# Autodesk Inventor assembly: Assembly1
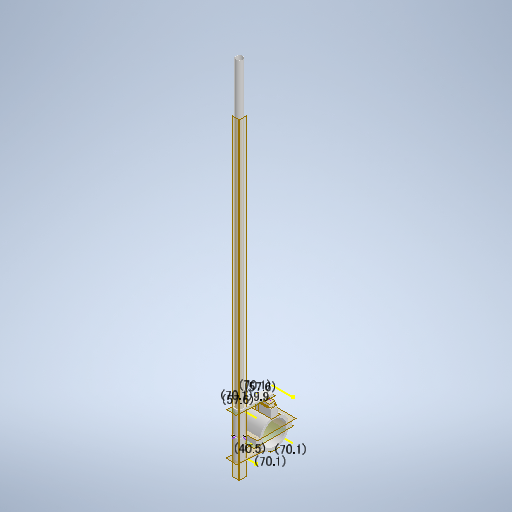
[picture p0: Inventor's stored thumbnail of the model, 512x512]
Saved by Autodesk Inventor 2025.2 (Build 292293000, 293)
## iProperties
Created: 2024-12-15
Part Number: Assembly1
Document SubType Name: Assembly
Designer: mahhy
Mass: 1247.47 g
Surface Area: 2591.78 cm^2
Volume: 1247.47 cm^3
Density: 1 g/cm^3
Author: mahhy
## Documents named in this file (15)
- D:\兵庫県立大\鳥人間部\尾翼データ\Assembly1.iam
- D:\兵庫県立大\鳥人間部\尾翼データ\motor_mount1.ipt
- D:\兵庫県立大\鳥人間部\尾翼データ\motor_mount2.ipt
- D:\兵庫県立大\鳥人間部\尾翼データ\wing1.ipt
- D:\兵庫県立大\鳥人間部\尾翼データ\bearing.ipt
- D:\兵庫県立大\鳥人間部\尾翼データ\arm1.ipt
- D:\兵庫県立大\鳥人間部\尾翼データ\arm2.ipt
- D:\兵庫県立大\鳥人間部\尾翼データ\servo_motor.ipt
- D:\兵庫県立大\鳥人間部\尾翼データ\pole.ipt
- D:\兵庫県立大\鳥人間部\尾翼データ\Assembly1\AIP\FEA\ewx9ztyo0.fins
- D:\兵庫県立大\鳥人間部\尾翼データ\Assembly1\AIP\FEA\ewx9ztyo0.fsat
- D:\兵庫県立大\鳥人間部\尾翼データ\Assembly1\AIP\FEA\ewx9ztyo0.ftes
- D:\兵庫県立大\鳥人間部\尾翼データ\Assembly1\AIP\FEA\ewx9ztyo0.fwiz
- D:\兵庫県立大\鳥人間部\尾翼データ\Assembly1\AIP\FEA\ewx9ztyrk.fmsh
- D:\兵庫県立大\鳥人間部\尾翼データ\Assembly1\AIP\FEA\ewx9ztyrl.fres
## Components (8 placed, 8 different names)
1. motor_mount1:1 — リジッド:1, リジッド:2
2. motor_mount2:1 — リジッド:1, 挿入:4
3. wing1:1 — 挿入:3, 挿入:5
4. bearing:1 — 挿入:1, 挿入:4
5. arm1:2 — 挿入:3, メイト:1
6. arm2:2 — 挿入:1, メイト:2, 挿入:6
7. servo_motor:1 — リジッド:2, 挿入:5
8. pole:1 — 挿入:6
## Relationships (10: Insert 5, Mate 3, WeldJoint 2)
- リジッド:1 [WeldJoint]: motor_mount1:1 ↔ motor_mount2:1
- 挿入:1 [Insert]: bearing:1 ↔ arm2:2
- リジッド:2 [WeldJoint]: motor_mount1:1 ↔ servo_motor:1
- 挿入:3 [Insert]: wing1:1 ↔ arm1:2
- 挿入:4 [Insert]: motor_mount2:1 ↔ bearing:1
- 挿入:5 [Insert]: wing1:1 ↔ servo_motor:1
- メイト:1 [Mate]: arm1:2
- メイト:2 [Mate]: arm2:2
- メイト:3 [Mate]
- 挿入:6 [Insert]: arm2:2 ↔ pole:1
## Named parameters: sa_0 = 10000, sa_1 = 0 mm, sa_2 = 0 mm, sa_3 = 0 mm
note: some values were not read from the file. Shown as the stored number, unit unknown: "sa_0".
